# Autodesk Inventor assembly: vp6242
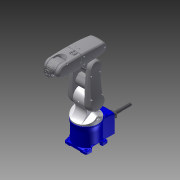
[picture p0: Inventor's stored thumbnail of the model, 180x180]
Saved by Autodesk Inventor 2013 (Build 170138000, 138)
## iProperties
Created: 2013-01-29
Part Number: vp6242
Document SubType Name: Assembly
Designer: Mahisorn
Author: Mahisorn
## Documents named in this file (7)
- E:\mahisorn\documents\hg-ros-pkg\cad\gripper\vp6242.iam
- E:\mahisorn\documents\hg-ros-pkg\cad\gripper\Imported Components\410590-0170-c001_drx\410590-0170-c001_drx.ipt
- E:\mahisorn\documents\hg-ros-pkg\cad\gripper\Imported Components\410590-0170-c002_drx\410590-0170-c002_drx.ipt
- E:\mahisorn\documents\hg-ros-pkg\cad\gripper\Imported Components\410590-0170-c003_drx\410590-0170-c003_drx.ipt
- E:\mahisorn\documents\hg-ros-pkg\cad\gripper\Imported Components\410590-0170-c004_drx\410590-0170-c004_drx.ipt
- E:\mahisorn\documents\hg-ros-pkg\cad\gripper\Imported Components\410590-0170-c005_drx\410590-0170-c005_drx.ipt
- E:\mahisorn\documents\hg-ros-pkg\cad\gripper\Imported Components\410590-0170-c006_drx\410590-0170-c006_drx.ipt
## Components (6 placed, 6 different names)
1. 410590-0170-c001_drx:1 — Insert:1
2. 410590-0170-c002_drx:1 — Insert:1, Insert:2
3. 410590-0170-c003_drx:1 — Insert:2, Insert:3
4. 410590-0170-c004_drx:1 — Insert:3, Insert:4
5. 410590-0170-c005_drx:1 — Insert:4, Insert:5
6. 410590-0170-c006_drx:1 — Insert:5
## Relationships (5: Insert 5)
- Insert:1: 410590-0170-c001_drx:1 ↔ 410590-0170-c002_drx:1
- Insert:2: 410590-0170-c002_drx:1 ↔ 410590-0170-c003_drx:1
- Insert:3: 410590-0170-c003_drx:1 ↔ 410590-0170-c004_drx:1
- Insert:4: 410590-0170-c004_drx:1 ↔ 410590-0170-c005_drx:1
- Insert:5: 410590-0170-c005_drx:1 ↔ 410590-0170-c006_drx:1
